# Autodesk Inventor assembly: Battery Cage Assembly
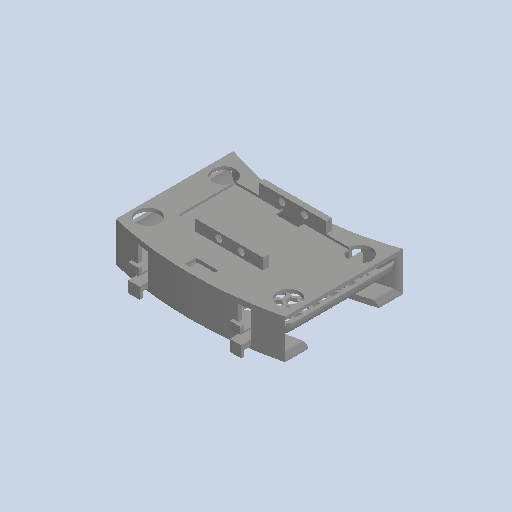
[picture p0: Inventor's stored thumbnail of the model, 512x512]
Saved by Autodesk Inventor 2023 (Build 270158000, 158)
## iProperties
Created: 2023-03-05
Part Number: Battery Cage Assembly
Document SubType Name: Assembly
Designer: cheng
Mass: 145.024 g
Surface Area: 985.289 cm^2
Volume: 116.017 cm^3
Density: 1.25002 g/cm^3
Author: cheng
## Documents named in this file (3)
- C:\Users\mihal\Desktop\4th Year Project\Final Assembly\Battery Cage and Sprind Plate\Battery Cage Assembly.iam
- C:\Users\mihal\Desktop\4th Year Project\Final Assembly\Battery Cage and Sprind Plate\Spring Plate.ipt
- C:\Users\mihal\Desktop\4th Year Project\Final Assembly\Battery Cage and Sprind Plate\Battery Cage.ipt
## Components (2 placed, 2 different names)
1. Spring Plate:1 — Mate:2, Mate:3
2. Battery Cage:1 — Mate:2, Mate:3
## Relationships (2: Mate 2)
- Mate:2: Spring Plate:1 ↔ Battery Cage:1
- Mate:3 (15 mm): Spring Plate:1 ↔ Battery Cage:1
